# Autodesk Inventor assembly: Bulldog Feeder
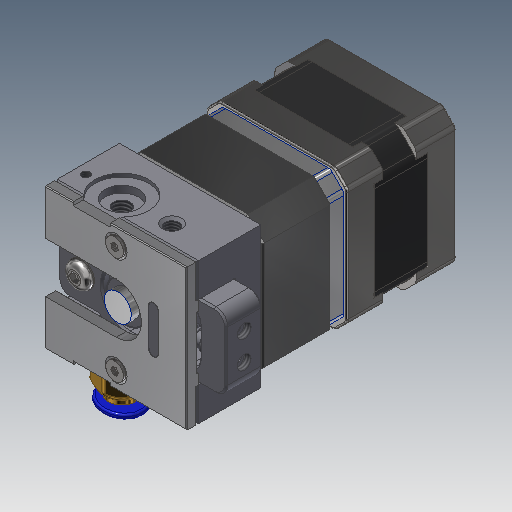
[picture p0: Inventor's stored thumbnail of the model, 512x512]
Saved by Autodesk Inventor 2017 (Build 210142000, 142)
## iProperties
Company: FABLAB Frenchmakers
Part Number: Bulldog Feeder
Material: Générique
Document SubType Name: Assembly
Designer: FABLAB Frenchmakers
Mass: 266.719 g
Surface Area: 599.862 cm^2
Volume: 116.534 cm^3
Density: 2.28877 g/cm^3
Project: 1420 Vauban 3D XL
Catalog Web Link: http://frenchmakers.com/
Stock Number: 1420-05-10
## Documents named in this file (14)
- W:\Professionnel\Conception FABLAB\1420-Vauban 3D XL\1420-05 Feeder\1420-05-10 Bulldog feeder.iam
- W:\Professionnel\Conception FABLAB\1420-Vauban 3D XL\1420-05 Feeder\1420-05-20 Nema 17 H30.ipt
- W:\Professionnel\Conception FABLAB\1420-Vauban 3D XL\1420-05 Feeder\1420-05-11 Reducteur.ipt
- W:\Professionnel\Conception FABLAB\1420-Vauban 3D XL\1420-05 Feeder\1420-05-12 Cache reducteur.ipt
- W:\Professionnel\Conception FABLAB\1420-Vauban 3D XL\1420-05 Feeder\1420-05-14 Support coulisse.ipt
- W:\Professionnel\Conception FABLAB\1420-Vauban 3D XL\1420-05 Feeder\1420-05-15 Coulisse.ipt
- W:\Professionnel\Conception FABLAB\1420-Vauban 3D XL\1420-05 Feeder\1420-05-18 Ressort.ipt
- W:\Professionnel\Conception FABLAB\1420-Vauban 3D XL\1420-05 Feeder\1420-05-21 M5 pour ressort.ipt
- W:\Professionnel\Conception FABLAB\1420-Vauban 3D XL\1420-05 Feeder\1420-05-17 Roulement a bille 634ZZ.ipt
- W:\Professionnel\Conception FABLAB\1420-Vauban 3D XL\1420-05 Feeder\1420-05-13 Roue dente.ipt
- W:\Professionnel\Conception FABLAB\1420-Vauban 3D XL\1420-90 Centre de contenu\fr-FR\ANSI B18.3.4M(1)\ANSI B18.3.4M - M4 x 0.7 x 16(2).ipt
- W:\Professionnel\Conception FABLAB\1420-Vauban 3D XL\1420-05 Feeder\1420-05-16 Plaque de maintient.ipt
- W:\Professionnel\Conception FABLAB\1420-Vauban 3D XL\1420-05 Feeder\1420-05-19 Clip pneumatique.ipt
- W:\Professionnel\Conception FABLAB\1420-Vauban 3D XL\1420-90 Centre de contenu\fr-FR\ASME ANSI B18.3.5M(2)\ASME_ANSI B18.3.5M - M3x6(2).ipt
## Components (16 placed, 13 different names)
1. 1420-05-20 Nema 17 H30:1 — Placage:1, Placage:2, Placage:3, Angle:1
2. 1420-05-11 Reducteur:1 — Placage:1, Placage:2, Placage:3, Placage:4, Placage:5, Placage:6, Placage:17, Affleurement:4
3. 1420-05-12 Cache reducteur:1 — Placage:4, Angle:1, Placage:5, Placage:7, Angle:2
4. 1420-05-14 Support coulisse:1 — Placage:6, Placage:7, Angle:2, Placage:8, Placage:9, Placage:10, Placage:11, Affleurement:2, Placage:12, Placage:13, Placage:16, Placage:20, Placage:21, Placage:22, Placage:27, Placage:28, Logement:1
5. 1420-05-15 Coulisse:1 — Placage:8, Placage:9, Placage:15, Placage:18, Placage:19
6. 1420-05-18 Ressort:1 — Placage:10, Affleurement:1, Affleurement:2
7. 1420-05-18 Ressort:2 — Placage:11, Affleurement:1, Placage:14
8. 1420-05-21 M5 pour ressort:1 — Affleurement:3, Placage:13
9. 1420-05-21 M5 pour ressort:2 — Affleurement:3, Placage:12, Placage:14
10. 1420-05-17 Roulement a bille 634ZZ:1 — Placage:15, Placage:16
11. 1420-05-13 Roue dente:1 — Placage:17, Affleurement:4
12. Vis percée à tête bombée à six pans creux - Métrique M4 x 0.7 x 16:1 — Placage:18, Placage:19
13. 1420-05-16 Plaque de maintient:1 — Placage:20, Placage:21, Placage:22, Placage:29
14. 1420-05-19 Clip pneumatique:2 — Logement:1
15. Vis percées à tête fraisée plate à six pans creux - Série métrique M3x6:1 — Placage:27, Affleurement:5, Placage:29
16. Vis percées à tête fraisée plate à six pans creux - Série métrique M3x6:2 — Placage:28, Affleurement:5
## Relationships (33: Mate 25, Flush 5, Angle 2, Insert 1)
- Placage:1 [Mate]: 1420-05-20 Nema 17 H30:1 ↔ 1420-05-11 Reducteur:1
- Placage:2 [Mate]: 1420-05-20 Nema 17 H30:1 ↔ 1420-05-11 Reducteur:1
- Placage:3 [Mate]: 1420-05-20 Nema 17 H30:1 ↔ 1420-05-11 Reducteur:1
- Placage:4 [Mate]: 1420-05-11 Reducteur:1 ↔ 1420-05-12 Cache reducteur:1
- Angle:1 (0 deg): 1420-05-20 Nema 17 H30:1 ↔ 1420-05-12 Cache reducteur:1
- Placage:5 [Mate]: 1420-05-11 Reducteur:1 ↔ 1420-05-12 Cache reducteur:1
- Placage:6 [Mate]: 1420-05-11 Reducteur:1 ↔ 1420-05-14 Support coulisse:1
- Placage:7 [Mate]: 1420-05-12 Cache reducteur:1 ↔ 1420-05-14 Support coulisse:1
- Angle:2 (0 deg): 1420-05-12 Cache reducteur:1 ↔ 1420-05-14 Support coulisse:1
- Placage:8 [Mate]: 1420-05-14 Support coulisse:1 ↔ 1420-05-15 Coulisse:1
- Placage:9 [Mate]: 1420-05-14 Support coulisse:1 ↔ 1420-05-15 Coulisse:1
- Placage:10 [Mate]: 1420-05-14 Support coulisse:1 ↔ 1420-05-18 Ressort:1
- Placage:11 [Mate]: 1420-05-14 Support coulisse:1 ↔ 1420-05-18 Ressort:2
- Affleurement:1 [Flush]: 1420-05-18 Ressort:1 ↔ 1420-05-18 Ressort:2
- Affleurement:2 [Flush]: 1420-05-14 Support coulisse:1 ↔ 1420-05-18 Ressort:1
- Affleurement:3 [Flush]: 1420-05-21 M5 pour ressort:1 ↔ 1420-05-21 M5 pour ressort:2
- Placage:12 [Mate]: 1420-05-14 Support coulisse:1 ↔ 1420-05-21 M5 pour ressort:2
- Placage:13 [Mate]: 1420-05-14 Support coulisse:1 ↔ 1420-05-21 M5 pour ressort:1
- Placage:14 [Mate]: 1420-05-18 Ressort:2 ↔ 1420-05-21 M5 pour ressort:2
- Placage:15 [Mate]: 1420-05-15 Coulisse:1 ↔ 1420-05-17 Roulement a bille 634ZZ:1
- Placage:16 [Mate]: 1420-05-14 Support coulisse:1 ↔ 1420-05-17 Roulement a bille 634ZZ:1
- Placage:17 [Mate]: 1420-05-11 Reducteur:1 ↔ 1420-05-13 Roue dente:1
- Affleurement:4 [Flush] (2.5 mm): 1420-05-11 Reducteur:1 ↔ 1420-05-13 Roue dente:1
- Placage:18 [Mate]: 1420-05-15 Coulisse:1 ↔ Vis percée à tête bombée à six pans creux - Métrique M4 x 0.7 x 16:1
- Placage:19 [Mate]: 1420-05-15 Coulisse:1 ↔ Vis percée à tête bombée à six pans creux - Métrique M4 x 0.7 x 16:1
- Placage:20 [Mate]: 1420-05-14 Support coulisse:1 ↔ 1420-05-16 Plaque de maintient:1
- Placage:21 [Mate]: 1420-05-14 Support coulisse:1 ↔ 1420-05-16 Plaque de maintient:1
- Placage:22 [Mate]: 1420-05-14 Support coulisse:1 ↔ 1420-05-16 Plaque de maintient:1
- Placage:27 [Mate]: 1420-05-14 Support coulisse:1 ↔ Vis percées à tête fraisée plate à six pans creux - Série métrique M3x6:1
- Placage:28 [Mate]: 1420-05-14 Support coulisse:1 ↔ Vis percées à tête fraisée plate à six pans creux - Série métrique M3x6:2
- Affleurement:5 [Flush]: Vis percées à tête fraisée plate à six pans creux - Série métrique M3x6:1 ↔ Vis percées à tête fraisée plate à six pans creux - Série métrique M3x6:2
- Placage:29 [Mate]: 1420-05-16 Plaque de maintient:1 ↔ Vis percées à tête fraisée plate à six pans creux - Série métrique M3x6:1
- Logement:1 [Insert]: 1420-05-14 Support coulisse:1 ↔ 1420-05-19 Clip pneumatique:2
